# Autodesk Inventor assembly: cycloid_assy
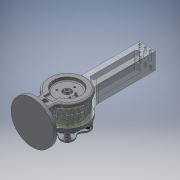
[picture p0: Inventor's stored thumbnail of the model, 180x180]
Saved by Autodesk Inventor 2019.3 (Build 233278000, 278)
## iProperties
Created: 2019-08-28
Part Number: cycloid_assy
Document SubType Name: Assembly
Designer: cdi
Author: cdi
## Documents named in this file (17)
- C:\Users\cdi\SynologyDrive\workspace_inventor\2019_06_19.MT4008_actuator\cycloid_gear_design_v1\cycloid_assy.iam
- C:\Users\cdi\SynologyDrive\workspace_inventor\2019_06_19.MT4008_actuator\cycloid_gear_design_v1\bearing_27x20x4.ipt
- C:\Users\cdi\SynologyDrive\workspace_inventor\2019_06_19.MT4008_actuator\cycloid_gear_design_v1\cycloid_base.ipt
- C:\Users\cdi\SynologyDrive\workspace_inventor\2019_06_19.MT4008_actuator\cycloid_gear_design_v1\rod_3x25.ipt
- C:\Users\cdi\SynologyDrive\workspace_inventor\2019_06_19.MT4008_actuator\cycloid_gear_design_v1\bearing_65x50x7.ipt
- C:\Users\cdi\SynologyDrive\workspace_inventor\2019_06_19.MT4008_actuator\cycloid_gear_design_v1\bearing_18x12x4.ipt
- C:\Users\cdi\SynologyDrive\workspace_inventor\2019_06_19.MT4008_actuator\cycloid_gear_design_v1\cycloid_top_bottom_assy.iam
- C:\Users\cdi\SynologyDrive\workspace_inventor\2019_06_19.MT4008_actuator\tarot-mt4008-motor-1.snapshot.3\inventor_export\Tarot 4008 Motor Assembly.iam
- C:\Users\cdi\SynologyDrive\workspace_inventor\2019_06_19.MT4008_actuator\cycloid_gear_design_v1\cycloid_housing.ipt
- C:\Users\cdi\SynologyDrive\workspace_altium\190430_MJVESC_MINI_VER0.3\MJVESC_MINI_CIR\3D_Export\inv\MJVESC_MINI_VER03.ipt
- C:\Users\cdi\SynologyDrive\workspace_inventor\2019_06_19.MT4008_actuator\cycloid_gear_design_v1\cycloid_base_mc.ipt
- C:\Users\cdi\SynologyDrive\workspace_inventor\2019_06_19.MT4008_actuator\cycloid_gear_design_v1\cycloid_motor_fix_plate.ipt
- C:\Users\cdi\SynologyDrive\workspace_inventor\2019_06_19.MT4008_actuator\cycloid_gear_design_v1\cycloid_input_cam_assy.ipt.iam
- C:\Users\cdi\SynologyDrive\workspace_altium\180512_AS5147_ENC_VER0.1\3D_Export\Inventor_AS5147_ENC_ANGLE_VER01\AS5147_ENC_ANGLE_VER01.iam
- C:\Users\cdi\SynologyDrive\workspace_inventor\2019_06_19.MT4008_actuator\cycloid_gear_design_v1\as5047_holder_adder_5mm.ipt
- C:\Users\cdi\SynologyDrive\workspace_inventor\2019_06_19.MT4008_actuator\cycloid_gear_design_v1\cycloid_fixing_base.ipt
- cycloid_input_cam_assy.ipt
## Components (27 placed, 15 different names)
1. cycloid_base:1 — Mate:4, Mate:5, Mate:7, Mate:8, Mate:36, Mate:38, Mate:39, Mate:41, Mate:46, Angle:1, Mate:65, Mate:66, Mate:67, Mate:79, Mate:80
2. bearing_65x50x7:1 — Mate:7, Mate:8, Flush:3
3. bearing_65x50x7:2 — Flush:4, Mate:47, Mate:48
4. bearing_18x12x4:1 — Mate:56, Mate:57, Mate:58, Mate:59
5. bearing_27x20x4:2 — Mate:18, Mate:70, Flush:5
6. bearing_27x20x4:4 — Mate:18, Mate:36, Mate:63, Mate:71
7. bearing_27x20x4:6 — Mate:32, Mate:60, Mate:62
8. bearing_27x20x4:7 — Mate:32, Mate:61, Mate:72, Flush:6
9. Tarot 4008 Motor Assembly:1 [sub-assembly] — Mate:40, Mate:41, Mate:55
10. cycloid_housing:1 — Mate:38, Flush:3, Flush:4
11. MJVESC_MINI_VER03:1 — Mate:49, Mate:68
12. cycloid_base_mc:1 — Mate:47, Mate:48, Mate:49, Angle:1, Mate:57, Mate:58, Mate:65, Mate:73, Mate:75, Mate:77, Mate:78
13. cycloid_motor_fix_plate:1 — Mate:55, Mate:66, Mate:67
14. cycloid_input_cam_assy.ipt:1 [sub-assembly] — Mate:56, Mate:59, Mate:60, Mate:61, Mate:62, Mate:63, Mate:68, Mate:70
15. cycloid_top_bottom_assy:3 [sub-assembly] — Mate:71, Tangent:2, Flush:5
16. cycloid_top_bottom_assy:4 [sub-assembly] — Mate:72, Tangent:1, Flush:6
17. AS5147_ENC_ANGLE_VER01:1 [sub-assembly] — Mate:74, Mate:76
18. as5047_holder_adder_5mm:1 — Mate:73, Mate:74, Mate:75, Mate:76, Mate:77
19. cycloid_fixing_base:1 — Mate:78, Mate:79, Mate:80
20. rod_3x25:1 — Mate:4, Mate:5
21. rod_3x25:2
22. rod_3x25:3 — Tangent:1
23. rod_3x25:4
24. rod_3x25:5 — Tangent:2
25. rod_3x25:6
26. rod_3x25:7
27. rod_3x25:8
## Component patterns: (8 elements, first: rod_3x25:1)
## Relationships (46: Mate 39, Flush 4, Tangent 2, Angle 1)
- Mate:4: cycloid_base:1 ↔ rod_3x25:1
- Mate:5: cycloid_base:1 ↔ rod_3x25:1
- Mate:7: cycloid_base:1 ↔ bearing_65x50x7:1
- Mate:8: cycloid_base:1 ↔ bearing_65x50x7:1
- Mate:18: bearing_27x20x4:2 ↔ bearing_27x20x4:4
- Mate:32: bearing_27x20x4:6 ↔ bearing_27x20x4:7
- Mate:36 (0.5 mm): cycloid_base:1 ↔ bearing_27x20x4:4
- Mate:38: cycloid_base:1 ↔ cycloid_housing:1
- Flush:3: bearing_65x50x7:1 ↔ cycloid_housing:1
- Flush:4: bearing_65x50x7:2 ↔ cycloid_housing:1
- Mate:39: cycloid_base:1
- Mate:40: Tarot 4008 Motor Assembly:1
- Mate:41: cycloid_base:1 ↔ Tarot 4008 Motor Assembly:1
- Mate:46: cycloid_base:1
- Mate:47: bearing_65x50x7:2 ↔ cycloid_base_mc:1
- Mate:48: bearing_65x50x7:2 ↔ cycloid_base_mc:1
- Mate:49: MJVESC_MINI_VER03:1 ↔ cycloid_base_mc:1
- Angle:1 (0 deg): cycloid_base:1 ↔ cycloid_base_mc:1
- Mate:55: Tarot 4008 Motor Assembly:1 ↔ cycloid_motor_fix_plate:1
- Mate:56: bearing_18x12x4:1 ↔ cycloid_input_cam_assy.ipt:1
- Mate:57: bearing_18x12x4:1 ↔ cycloid_base_mc:1
- Mate:58: bearing_18x12x4:1 ↔ cycloid_base_mc:1
- Mate:59: bearing_18x12x4:1 ↔ cycloid_input_cam_assy.ipt:1
- Mate:60: bearing_27x20x4:6 ↔ cycloid_input_cam_assy.ipt:1
- Mate:61: bearing_27x20x4:7 ↔ cycloid_input_cam_assy.ipt:1
- Mate:62: bearing_27x20x4:6 ↔ cycloid_input_cam_assy.ipt:1
- Mate:63: bearing_27x20x4:4 ↔ cycloid_input_cam_assy.ipt:1
- Mate:65: cycloid_base:1 ↔ cycloid_base_mc:1
- Mate:66: cycloid_base:1 ↔ cycloid_motor_fix_plate:1
- Mate:67: cycloid_base:1 ↔ cycloid_motor_fix_plate:1
- Mate:68: MJVESC_MINI_VER03:1 ↔ cycloid_input_cam_assy.ipt:1
- Mate:70: bearing_27x20x4:2 ↔ cycloid_input_cam_assy.ipt:1
- Mate:71: bearing_27x20x4:4 ↔ cycloid_top_bottom_assy:3
- Mate:72: bearing_27x20x4:7 ↔ cycloid_top_bottom_assy:4
- Tangent:1: cycloid_top_bottom_assy:4 ↔ rod_3x25:3
- Tangent:2: cycloid_top_bottom_assy:3 ↔ rod_3x25:5
- Flush:5: bearing_27x20x4:2 ↔ cycloid_top_bottom_assy:3
- Flush:6: bearing_27x20x4:7 ↔ cycloid_top_bottom_assy:4
- Mate:73: cycloid_base_mc:1 ↔ as5047_holder_adder_5mm:1
- Mate:74: AS5147_ENC_ANGLE_VER01:1 ↔ as5047_holder_adder_5mm:1
- Mate:75: cycloid_base_mc:1 ↔ as5047_holder_adder_5mm:1
- Mate:76: AS5147_ENC_ANGLE_VER01:1 ↔ as5047_holder_adder_5mm:1
- Mate:77: cycloid_base_mc:1 ↔ as5047_holder_adder_5mm:1
- Mate:78: cycloid_base_mc:1 ↔ cycloid_fixing_base:1
- Mate:79: cycloid_base:1 ↔ cycloid_fixing_base:1
- Mate:80: cycloid_base:1 ↔ cycloid_fixing_base:1
